# Autodesk Inventor assembly: Шотер_В5
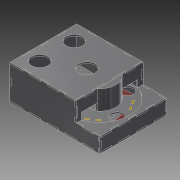
[picture p0: Inventor's stored thumbnail of the model, 180x180]
Saved by Autodesk Inventor 2022 (Build 260153000, 153)
## iProperties
Part Number: Шотер_В5
Checked By: Якушев
Engr Approved By: Малов
Material: Типовые
Document SubType Name: Assembly
Mfg Approved By: Судаков
Designer: Смирнов
Author: Смирнов
## Documents named in this file (3)
- E:\4. Прочее\1517\Предпрофессиональная олимпиада\Shoter_V5\Шотер_В5.iam
- E:\4. Прочее\1517\Предпрофессиональная олимпиада\Shoter_V5\Корпус_В5_исходник.ipt
- E:\4. Прочее\1517\Предпрофессиональная олимпиада\Shoter_V5\Поворотный_модуль_В5.iam
## Components (2 placed, 2 different names)
1. Корпус_В5_исходник:1 — Совмещение:1, Совмещение:2
2. Поворотный_модуль_В5:1 [sub-assembly] — Совмещение:1, Совмещение:2
## Relationships (2: Mate 2)
- Совмещение:1 [Mate]: Корпус_В5_исходник:1 ↔ Поворотный_модуль_В5:1
- Совмещение:2 [Mate] (2 mm): Корпус_В5_исходник:1 ↔ Поворотный_модуль_В5:1
